# Autodesk Inventor assembly: Gripper
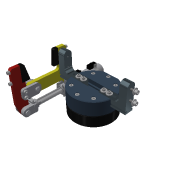
[picture p0: Inventor's stored thumbnail of the model, 180x180]
Saved by Autodesk Inventor 2020.1 (Build 241239000, 239)
## iProperties
Created: 2006-01-31
Part Number: Gripper
Document SubType Name: Assembly
Designer: Kevin
Manufacturer: Standard
Standards Organization: Custom
Weld Material: Default
Author: Kevin
Revision Number: -
## Documents named in this file (13)
- C:\Users\thom_tremblay\Desktop\Inventor ACP Data\Gripper - Structure.iam
- C:\Users\thom_tremblay\Desktop\Inventor ACP Data\Parts\210-100.ipt
- C:\Users\thom_tremblay\Desktop\Inventor ACP Data\Parts\210-101ipt.ipt
- C:\Users\thom_tremblay\Desktop\Inventor ACP Data\Content Center\en-US\ISO 4762\M8-65.ipt
- C:\Users\thom_tremblay\Desktop\Inventor ACP Data\Content Center\en-US\ISO 4762\M6-45.ipt
- C:\Users\thom_tremblay\Desktop\Inventor ACP Data\Content Center\en-US\ISO 7089\10.ipt
- C:\Users\thom_tremblay\Desktop\Inventor ACP Data\Assemblies\210-103.iam
- C:\Users\thom_tremblay\Desktop\Inventor ACP Data\Assemblies\PH-000-001.iam
- C:\Users\thom_tremblay\Desktop\Inventor ACP Data\Content Center\en-US\ISO 4762\M8-30.ipt
- C:\Users\thom_tremblay\Desktop\Inventor ACP Data\Assemblies\PH-000-002.iam
- C:\Users\thom_tremblay\Desktop\Inventor ACP Data\Assemblies\210-110.IAM
- C:\Users\thom_tremblay\Desktop\Inventor ACP Data\Parts\210-102 f.ipt
- C:\Users\thom_tremblay\Desktop\Inventor ACP Data\Libraries\Simulation\Gripper_res_{3E676F27-C720-4572-8F7D-DA90B4A1A400}.fres
## Components (30 placed, 11 different names)
1. 210-100:1 — Mate:1, Insert:1
2. 210-101ipt:1 — Mate:1, Insert:1, Mate:2, Mate:6, Mate:25, Mate:26, Mate:27, Mate:28, Mate:29, Insert:21, Mate:36, Mate:37, Mate:38, Mate:3
3. 210-102 f:1 — Mate:2, Mate:3, Insert:36, Angle:3, Mate:42
4. 210-102 f:2 — Mate:25, Mate:26, Mate:29, Mate:41
5. 210-103:1 [sub-assembly] — Insert:19, Insert:31, Insert:34, Insert:30, Insert:36
6. 210-110:1 [sub-assembly] — Insert:34, Mate:40, Angle:3
7. PH-000-001:1 [sub-assembly] — Insert:19, Mate:32
8. PH-000-002:1 [sub-assembly] — Mate:32, Mate:40
9. ISO 4762 M8 x 45:1 — Mate:6, Insert:22, Mate:42
10. ISO 7089 10 - 140 HV:1 — Insert:22
11. ISO 7089 10 - 140 HV:2 — Insert:23
12. ISO 4762 M8 x 45:2 — Insert:23, Mate:36
13. ISO 7089 10 - 140 HV:3 — Mate:28, Insert:25
14. ISO 4762 M8 x 45:3 — Insert:25, Mate:38
15. ISO 7089 10 - 140 HV:4 — Mate:27, Insert:24
16. ISO 4762 M8 x 45:4 — Mate:37, Insert:24
17. ISO 7089 10 - 140 HV:5 — Insert:33, Insert:30
18. ISO 7089 10 - 140 HV:6 — Insert:31, Insert:32
19. ISO 7089 10 - 140 HV:7 — Insert:28
20. ISO 7089 10 - 140 HV:8 — Insert:29
21. ISO 4762 M8 x 30:1 — Insert:29
22. ISO 4762 M8 x 30:2 — Insert:28, Mate:41
23. ISO 4762 M8 x 30:3 — Insert:32
24. ISO 4762 M8 x 30:4 — Insert:33
25. "ISO 4762 " M8 x 65:1 — Insert:21
26. "ISO 4762 " M8 x 65:2
27. "ISO 4762 " M8 x 65:3
28. "ISO 4762 " M8 x 65:4
29. "ISO 4762 " M8 x 65:5
30. "ISO 4762 " M8 x 65:6
## Component patterns: (8 elements, first: "ISO 4762 " M8 x 65:1)
## Relationships (35: Mate 19, Insert 15, Angle 1)
- Mate:1: 210-100:1 ↔ 210-101ipt:1
- Insert:1: 210-100:1 ↔ 210-101ipt:1
- Mate:2: 210-101ipt:1 ↔ 210-102 f:1
- [Mate]: 210-101ipt:1 ↔ 210-102 f:1
- Mate:6: 210-101ipt:1 ↔ ISO 4762 M8 x 45:1
- [Mate]: 210-102 f:2 ↔ ISO 7089 10 - 140 HV:1
- [Mate]: 210-101ipt:1 ↔ ISO 7089 10 - 140 HV:2
- Mate:25: 210-101ipt:1 ↔ 210-102 f:2
- Mate:26: 210-101ipt:1 ↔ 210-102 f:2
- Mate:27: 210-101ipt:1 ↔ ISO 7089 10 - 140 HV:4
- Mate:28: 210-101ipt:1 ↔ ISO 7089 10 - 140 HV:3
- Mate:29 (30 mm): 210-101ipt:1 ↔ 210-102 f:2
- Insert:19: 210-103:1 ↔ PH-000-001:1
- Mate:32: PH-000-001:1 ↔ PH-000-002:1
- Insert:21: 210-101ipt:1 ↔ "ISO 4762 " M8 x 65:1
- Insert:22: ISO 4762 M8 x 45:1 ↔ ISO 7089 10 - 140 HV:1
- Insert:23: ISO 7089 10 - 140 HV:2 ↔ ISO 4762 M8 x 45:2
- Mate:36: 210-101ipt:1 ↔ ISO 4762 M8 x 45:2
- Mate:37: 210-101ipt:1 ↔ ISO 4762 M8 x 45:4
- Insert:24: ISO 7089 10 - 140 HV:4 ↔ ISO 4762 M8 x 45:4
- Insert:25: ISO 7089 10 - 140 HV:3 ↔ ISO 4762 M8 x 45:3
- Mate:38: 210-101ipt:1 ↔ ISO 4762 M8 x 45:3
- Insert:28: ISO 7089 10 - 140 HV:7 ↔ ISO 4762 M8 x 30:2
- Insert:29: ISO 7089 10 - 140 HV:8 ↔ ISO 4762 M8 x 30:1
- Insert:31: 210-103:1 ↔ ISO 7089 10 - 140 HV:6
- Insert:32: ISO 7089 10 - 140 HV:6 ↔ ISO 4762 M8 x 30:3
- Insert:33: ISO 7089 10 - 140 HV:5 ↔ ISO 4762 M8 x 30:4
- Insert:34: 210-103:1 ↔ 210-110:1
- Mate:40: 210-110:1 ↔ PH-000-002:1
- Insert:30: 210-103:1 ↔ ISO 7089 10 - 140 HV:5
- Mate:3: 210-101ipt:1 ↔ 210-102 f:1
- Insert:36: 210-102 f:1 ↔ 210-103:1
- Angle:3 (0 deg): 210-102 f:1 ↔ 210-110:1
- Mate:41: 210-102 f:2 ↔ ISO 4762 M8 x 30:2
- Mate:42: 210-102 f:1 ↔ ISO 4762 M8 x 45:1
